# Autodesk Inventor assembly: frame
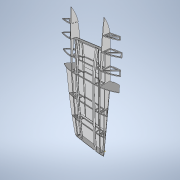
[picture p0: Inventor's stored thumbnail of the model, 180x180]
Saved by Autodesk Inventor 2020.3 (Build 243373010, 373A)
## iProperties
Created: 2020-05-22
Part Number: frame
Document SubType Name: Assembly
Designer: kardo
Mass: 169.879 g
Surface Area: 2584.8 cm^2
Volume: 169.879 cm^3
Density: 1 g/cm^3
Author: kardo
## Documents named in this file (16)
- D:\Computer Aided Design\hydroplane plan\frame.iam
- D:\Computer Aided Design\hydroplane plan\frame\stringer.ipt
- D:\Computer Aided Design\hydroplane plan\frame\bulkhead_main.ipt
- D:\Computer Aided Design\hydroplane plan\frame\bulkhead_F1.ipt
- D:\Computer Aided Design\hydroplane plan\frame\bulkhead_front.ipt
- D:\Computer Aided Design\hydroplane plan\frame\bulkhead_F2.ipt
- D:\Computer Aided Design\hydroplane plan\frame\bulkhead_B1.ipt
- D:\Computer Aided Design\hydroplane plan\frame\bulkhead_B2.ipt
- D:\Computer Aided Design\hydroplane plan\frame\transom.ipt
- D:\Computer Aided Design\hydroplane plan\frame\sidewall_rear.ipt
- D:\Computer Aided Design\hydroplane plan\frame\transom_plate.ipt
- D:\Computer Aided Design\hydroplane plan\frame\bottom_side_plate.ipt
- D:\Computer Aided Design\hydroplane plan\frame\bottom_offset_wall.ipt
- D:\Computer Aided Design\hydroplane plan\frame\bottom_offset_plate.ipt
- D:\Computer Aided Design\hydroplane plan\frame\cowl_strip.ipt
- D:\Computer Aided Design\hydroplane plan\frame\cowl_insulation.ipt
## Components (22 placed, 15 different names)
1. stringer:1 — Mate:5, Mate:6, Mate:7, Mate:16, Mate:17, Mate:19, Mate:51, Mate:54, Symmetry:1, Mate:73
2. stringer:2 — Mate:1, Mate:2, Mate:3, Mate:20, Mate:21, Mate:22, Mate:23, Mate:24, Mate:26, Mate:27, Mate:28, Mate:29, Mate:33, Mate:34, Mate:35, Mate:36, Mate:37, Mate:38, Mate:57, Mate:66, Mate:67, Mate:69, Symmetry:1
3. bulkhead_main:1 — Mate:1, Mate:2, Mate:3, Mate:5, Mate:6, Mate:7, Mate:62, Mate:63, Mate:74, Mate:75, Mate:76, Mate:77, Mate:78, Mate:79, Mate:80, Mate:81
4. bulkhead_F1:1 — Mate:23, Mate:27, Mate:28
5. bulkhead_front:1 — Mate:24, Mate:26, Mate:29, Mate:53, Mate:56, Mate:60, Mate:61
6. bulkhead_F2:1 — Mate:20, Mate:21, Mate:22
7. bulkhead_F2:2 — Mate:16, Mate:17, Mate:19
8. bulkhead_B1:1 — Mate:66, Mate:67, Mate:70
9. bulkhead_B2:1 — Mate:33, Mate:34, Mate:35, Mate:50
10. transom:1 — Mate:36, Mate:37, Mate:38, Mate:49, Mate:68, Mate:71
11. sidewall_rear:1 — Mate:68, Mate:69, Mate:70, Symmetry:2
12. sidewall_rear:2 — Symmetry:2, Mate:71, Mate:72
13. transom_plate:1 — Mate:49, Mate:50, Mate:51, Mate:52, Mate:55, Mate:58, Mate:59, Mate:65
14. bottom_side_plate:1 — Mate:55, Mate:56, Mate:57
15. bottom_side_plate:2 — Mate:52, Mate:53, Mate:54
16. bottom_offset_wall:1 — Mate:58, Mate:60, Mate:62, Mate:64
17. bottom_offset_wall:2 — Mate:59, Mate:61, Mate:63
18. bottom_offset_plate:1 — Mate:64, Mate:65
19. cowl_strip:1 — Mate:76, Mate:77
20. cowl_strip:2 — Mate:74, Mate:75
21. cowl_insulation:1 — Mate:78, Mate:79
22. cowl_insulation:2 — Mate:80, Mate:81
## Relationships (59: Mate 57, Symmetry 2)
- Mate:1: stringer:2 ↔ bulkhead_main:1
- Mate:2: stringer:2 ↔ bulkhead_main:1
- Mate:3: stringer:2 ↔ bulkhead_main:1
- Mate:5: stringer:1 ↔ bulkhead_main:1
- Mate:6: stringer:1 ↔ bulkhead_main:1
- Mate:7: stringer:1 ↔ bulkhead_main:1
- Mate:16: stringer:1 ↔ bulkhead_F2:2
- Mate:17: stringer:1 ↔ bulkhead_F2:2
- Mate:19: stringer:1 ↔ bulkhead_F2:2
- Mate:20: stringer:2 ↔ bulkhead_F2:1
- Mate:21: stringer:2 ↔ bulkhead_F2:1
- Mate:22: stringer:2 ↔ bulkhead_F2:1
- Mate:23: stringer:2 ↔ bulkhead_F1:1
- Mate:24: stringer:2 ↔ bulkhead_front:1
- Mate:26: stringer:2 ↔ bulkhead_front:1
- Mate:27: stringer:2 ↔ bulkhead_F1:1
- Mate:28: stringer:2 ↔ bulkhead_F1:1
- Mate:29: stringer:2 ↔ bulkhead_front:1
- Mate:33: stringer:2 ↔ bulkhead_B2:1
- Mate:34: stringer:2 ↔ bulkhead_B2:1
- Mate:35: stringer:2 ↔ bulkhead_B2:1
- Mate:36: stringer:2 ↔ transom:1
- Mate:37: stringer:2 ↔ transom:1
- Mate:38: stringer:2 ↔ transom:1
- Mate:49: transom:1 ↔ transom_plate:1
- Mate:50: bulkhead_B2:1 ↔ transom_plate:1
- Mate:51: stringer:1 ↔ transom_plate:1
- Mate:52: transom_plate:1 ↔ bottom_side_plate:2
- Mate:53: bulkhead_front:1 ↔ bottom_side_plate:2
- Mate:54: stringer:1 ↔ bottom_side_plate:2
- Mate:55: transom_plate:1 ↔ bottom_side_plate:1
- Mate:56: bulkhead_front:1 ↔ bottom_side_plate:1
- Mate:57: stringer:2 ↔ bottom_side_plate:1
- Mate:58: transom_plate:1 ↔ bottom_offset_wall:1
- Mate:59: transom_plate:1 ↔ bottom_offset_wall:2
- Mate:60: bulkhead_front:1 ↔ bottom_offset_wall:1
- Mate:61: bulkhead_front:1 ↔ bottom_offset_wall:2
- Mate:62: bulkhead_main:1 ↔ bottom_offset_wall:1
- Mate:63: bulkhead_main:1 ↔ bottom_offset_wall:2
- Mate:64: bottom_offset_wall:1 ↔ bottom_offset_plate:1
- Mate:65: transom_plate:1 ↔ bottom_offset_plate:1
- Mate:66: stringer:2 ↔ bulkhead_B1:1
- Mate:67: stringer:2 ↔ bulkhead_B1:1
- Mate:68: transom:1 ↔ sidewall_rear:1
- Mate:69: stringer:2 ↔ sidewall_rear:1
- Mate:70: bulkhead_B1:1 ↔ sidewall_rear:1
- Symmetry:1: stringer:1 ↔ stringer:2
- Symmetry:2: sidewall_rear:1 ↔ sidewall_rear:2
- Mate:71: transom:1 ↔ sidewall_rear:2
- Mate:72: sidewall_rear:2
- Mate:73: stringer:1
- Mate:74: bulkhead_main:1 ↔ cowl_strip:2
- Mate:75: bulkhead_main:1 ↔ cowl_strip:2
- Mate:76: bulkhead_main:1 ↔ cowl_strip:1
- Mate:77: bulkhead_main:1 ↔ cowl_strip:1
- Mate:78: bulkhead_main:1 ↔ cowl_insulation:1
- Mate:79: bulkhead_main:1 ↔ cowl_insulation:1
- Mate:80: bulkhead_main:1 ↔ cowl_insulation:2
- Mate:81: bulkhead_main:1 ↔ cowl_insulation:2
